# Autodesk Inventor assembly: cover1
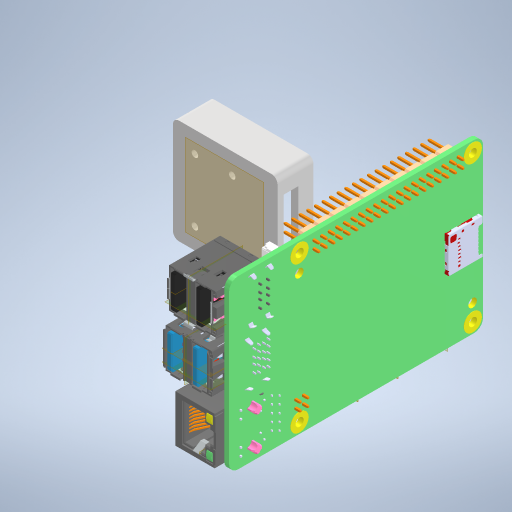
[picture p0: Inventor's stored thumbnail of the model, 512x512]
Saved by Autodesk Inventor 2024 (Build 280153000, 153)
## iProperties
Created: 2024-05-03
Part Number: cover1
Document SubType Name: Assembly
Designer: Pintu
Author: Pintu
## Documents named in this file (4)
- D:\CMC\my_inventor\ArmBo_v2\rpi\cover1.iam
- D:\CMC\my_inventor\ArmBo_v2\rpi\camera\Camera_module_3_wide_model_simple.iam
- D:\CMC\my_inventor\ArmBo_v2\rpi\cover_part.ipt
- D:\CMC\my_inventor\ArmBo_v2\rpi\rpi5\RASPBERRY_PI_5.iam
## Components (3 placed, 3 different names)
1. Camera_module_3_wide_model_simple:1 [sub-assembly] — Mate:1, Mate:2
2. cover_part:1 — Mate:1, Mate:2
3. RASPBERRY_PI_5:1 [sub-assembly]
## Relationships (2: Mate 2)
- Mate:1: Camera_module_3_wide_model_simple:1 ↔ cover_part:1
- Mate:2: Camera_module_3_wide_model_simple:1 ↔ cover_part:1
